# Autodesk Inventor assembly: Shooter Assembly
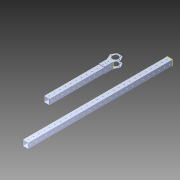
[picture p0: Inventor's stored thumbnail of the model, 180x180]
Saved by Autodesk Inventor 2014 (Build 180170000, 170)
## iProperties
Created: 2014-01-05
Part Number: Shooter Assembly
Document SubType Name: Assembly
Designer: Andrew Toennies
Author: Andrew Toennies
## Documents named in this file (4)
- C:\Users\Andrew Toennies\Documents\GitHub\2014buildCAD\Shooter\Shooter Assembly.iam
- C:\Users\Andrew Toennies\Documents\GitHub\2014buildCAD\Shooter\Vex Pro 1x1 rectangular tubing 12 in length.ipt
- C:\Users\Andrew Toennies\Documents\GitHub\2014buildCAD\Shooter\Vex Pro End Bearing Mount.ipt
- C:\Users\Andrew Toennies\Documents\GitHub\2014buildCAD\Shooter\Vex Pro 1x1 rectangular tubing 27 in length.ipt
## Components (4 placed, 3 different names)
1. Vex Pro 1x1 rectangular tubing 12 in length:1 — Insert:1, Insert:2, Insert:3, Insert:4
2. Vex Pro End Bearing Mount:1 — Insert:1, Insert:2
3. Vex Pro End Bearing Mount:2 — Insert:3, Insert:4
4. Vex Pro 1x1 rectangular tubing 27 in length:1
## Relationships (4: Insert 4)
- Insert:1: Vex Pro 1x1 rectangular tubing 12 in length:1 ↔ Vex Pro End Bearing Mount:1
- Insert:2: Vex Pro 1x1 rectangular tubing 12 in length:1 ↔ Vex Pro End Bearing Mount:1
- Insert:3: Vex Pro 1x1 rectangular tubing 12 in length:1 ↔ Vex Pro End Bearing Mount:2
- Insert:4: Vex Pro 1x1 rectangular tubing 12 in length:1 ↔ Vex Pro End Bearing Mount:2
